# Autodesk Inventor assembly: NEUROPIXELS GEN 2 PROBE ASSY
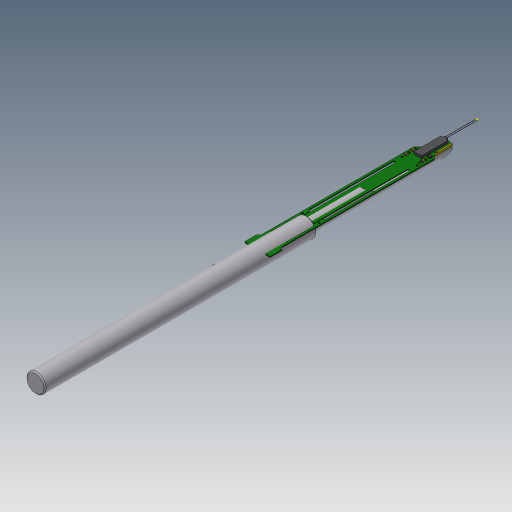
[picture p0: Inventor's stored thumbnail of the model, 512x512]
Saved by Autodesk Inventor 2023.4 (Build 274418000, 418)
## iProperties
RuleStatus: InUse
AfterDocSave0: file://Part Number Cleaner
Created: 2019-07-02
Vendor: HHMI: JRC - ID&F
Document SubType Name: Assembly
Designer: arnoldj
DESIGN DEPARTMENT: HHMI: JRC - ID&F
ALTERED ITEM PART NUMBER: N/A
ALTERED ITEM VENDOR: N/A
ALTERED ITEM DESCRIPTION: N/A
Author: arnoldj
Revision Number: 0
## Documents named in this file (6)
- C:\_WORKSPACE\DATA\PROJECTS\PROBE MOUNTS\MCAD\NEUROPIXELS GEN 2 PROBE ASSY.iam
- C:\_WORKSPACE\DATA\PROJECTS\PROBE MOUNTS\MCAD\NPM_FLEX_00-00.ipt
- C:\_WORKSPACE\DATA\PROJECTS\PROBE MOUNTS\MCAD\NEUROPIXELS DOVE TAIL MOUNT GEN 2.ipt
- C:\_WORKSPACE\DATA\PROJECTS\PROBE MOUNTS\MCAD\NEUROPIXELS GEN 2 DOVE TAIL PROBE HOLDER.ipt
- C:\_WORKSPACE\DATA\COMMON\Misumi\MISUMI_SSM-SUS-M1_6-2.ipt
- C:\_WORKSPACE\DATA\PROJECTS\PROBE MOUNTS\MCAD\NEUROPIXELS GEN 2 ROD ADAPTER.ipt
## Components (5 placed, 5 different names)
1. NEUROPIXELS GEN 2 DOVE TAIL PROBE HOLDER:1 — Mate:1, Mate:2, Flush:1, Flush:2, Mate:7, Mate:8, Mate:10, Mate:11
2. NEUROPIXELS DOVE TAIL MOUNT GEN 2:1 — Mate:1, Mate:2, Flush:1, Mate:3, Flush:3, Mate:7, Mate:9
3. NPM_FLEX_00-00:1 — Mate:3, Flush:2, Flush:3
4. MISUMI_SSM-SUS-M1_6-2:1 — Mate:8, Mate:9
5. NEUROPIXELS GEN 2 ROD ADAPTER:1 — Mate:10, Mate:11
## Relationships (11: Mate 8, Flush 3)
- Mate:1: NEUROPIXELS GEN 2 DOVE TAIL PROBE HOLDER:1 ↔ NEUROPIXELS DOVE TAIL MOUNT GEN 2:1
- Mate:2: NEUROPIXELS GEN 2 DOVE TAIL PROBE HOLDER:1 ↔ NEUROPIXELS DOVE TAIL MOUNT GEN 2:1
- Flush:1: NEUROPIXELS GEN 2 DOVE TAIL PROBE HOLDER:1 ↔ NEUROPIXELS DOVE TAIL MOUNT GEN 2:1
- Mate:3: NEUROPIXELS DOVE TAIL MOUNT GEN 2:1 ↔ NPM_FLEX_00-00:1
- Flush:2: NEUROPIXELS GEN 2 DOVE TAIL PROBE HOLDER:1 ↔ NPM_FLEX_00-00:1
- Flush:3: NEUROPIXELS DOVE TAIL MOUNT GEN 2:1 ↔ NPM_FLEX_00-00:1
- Mate:7: NEUROPIXELS GEN 2 DOVE TAIL PROBE HOLDER:1 ↔ NEUROPIXELS DOVE TAIL MOUNT GEN 2:1
- Mate:8: NEUROPIXELS GEN 2 DOVE TAIL PROBE HOLDER:1 ↔ MISUMI_SSM-SUS-M1_6-2:1
- Mate:9: NEUROPIXELS DOVE TAIL MOUNT GEN 2:1 ↔ MISUMI_SSM-SUS-M1_6-2:1
- Mate:10: NEUROPIXELS GEN 2 DOVE TAIL PROBE HOLDER:1 ↔ NEUROPIXELS GEN 2 ROD ADAPTER:1
- Mate:11: NEUROPIXELS GEN 2 DOVE TAIL PROBE HOLDER:1 ↔ NEUROPIXELS GEN 2 ROD ADAPTER:1
